# Autodesk Inventor assembly: super-shifter-asm-penumatic-hex-long
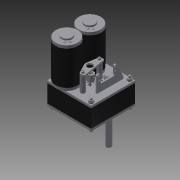
[picture p0: Inventor's stored thumbnail of the model, 180x180]
Saved by Autodesk Inventor 2014 (Build 180170000, 170)
## iProperties
Created: 2014-01-12
Part Number: super-shifter-asm-penumatic-hex-long
Document SubType Name: Assembly
Designer: Kelby
Author: Unknown
Title: //Amserv/amserver/AndyMark/Products/Gearboxes Shifters/Super Shifter/super-shifter-asm-penumatic-hex-long.stp
Organization: Unknown
Description: Unknown
Sending System: Unknown
Preprocessor: XStep 1.0
Author: Kelby
## Documents named in this file (7)
- C:\Users\Kelby\AppData\Local\Autodesk\Autodesk Sync\Cloud\brian.clegg5@gmail.com\Frc Chassis 2014\super-shifter-asm-penumatic-hex-long\super-shifter-asm-penumatic-hex-long.iam
- C:\Users\Kelby\AppData\Local\Autodesk\Autodesk Sync\Cloud\brian.clegg5@gmail.com\Frc Chassis 2014\super-shifter-asm-penumatic-hex-long\super_d10.ipt
- C:\Users\Kelby\AppData\Local\Autodesk\Autodesk Sync\Cloud\brian.clegg5@gmail.com\Frc Chassis 2014\super-shifter-asm-penumatic-hex-long\amshifter2_d02.ipt
- C:\Users\Kelby\AppData\Local\Autodesk\Autodesk Sync\Cloud\brian.clegg5@gmail.com\Frc Chassis 2014\super-shifter-asm-penumatic-hex-long\1-4-28_jam-nut.ipt
- C:\Users\Kelby\AppData\Local\Autodesk\Autodesk Sync\Cloud\brian.clegg5@gmail.com\Frc Chassis 2014\super-shifter-asm-penumatic-hex-long\10-32x2500_shcs.ipt
- C:\Users\Kelby\AppData\Local\Autodesk\Autodesk Sync\Cloud\brian.clegg5@gmail.com\Frc Chassis 2014\super-shifter-asm-penumatic-hex-long\super_shifter_asm-long-hex.iam
- C:\Users\Kelby\Desktop\Gearboxes\AM_ToughboxStandard\CIM motor.ipt
## Components (9 placed, 6 different names)
1. super_d10
2. super_d10:1
3. amshifter2_d02
4. 1-4-28_jam-nut
5. 10-32x2500_shcs
6. 10-32x2500_shcs:1
7. super_shifter_asm-long-hex [sub-assembly] — Insert:1, Insert:2
8. CIM motor:1 — Insert:1
9. CIM motor:2 — Insert:2
## Relationships (2: Insert 2)
- Insert:1: super_shifter_asm-long-hex ↔ CIM motor:1
- Insert:2: super_shifter_asm-long-hex ↔ CIM motor:2
